# Autodesk Inventor assembly: Assembly2
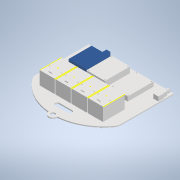
[picture p0: Inventor's stored thumbnail of the model, 180x180]
Saved by Autodesk Inventor 2020 (Build 240168000, 168)
## iProperties
Created: 2020-02-08
Part Number: Assembly2
Document SubType Name: Assembly
Designer: holtat
Author: holtat
## Documents named in this file (7)
- C:\Users\holtat\Documents\Inebriator\Assembly2.iam
- C:\Users\holtat\Documents\Inebriator\Top Plate.ipt
- C:\Users\holtat\Documents\Inebriator\Arduino.ipt
- C:\Users\holtat\Documents\Inebriator\ConnecterBoard.ipt
- C:\Users\holtat\Documents\Inebriator\Relay Board.ipt
- C:\Users\holtat\Documents\Inebriator\Plug.ipt
- C:\Users\holtat\Documents\Inebriator\Pump.ipt
## Components (9 placed, 6 different names)
1. Top Plate:1 — Mate:1, Mate:2, Mate:3, Mate:4, Mate:5, Mate:6, Flush:2, Flush:3, Flush:4, Flush:7, Mate:10, Flush:8, Mate:11, Flush:10
2. Arduino:1 — Mate:1, Flush:4, Mate:7, Flush:7
3. ConnecterBoard:1 — Mate:3, Flush:3, Mate:8
4. Relay Board:1 — Mate:2, Flush:2, Mate:7, Mate:8
5. Plug:1 — Mate:10, Flush:8
6. Pump:1 — Mate:6, Flush:6, Flush:9, Mate:13, Mate:14
7. Pump:2 — Mate:5, Flush:5, Flush:6, Mate:12, Flush:10
8. Pump:3 — Mate:4, Flush:5, Mate:12, Mate:13
9. Pump:4 — Mate:11, Flush:9, Mate:14
## Relationships (22: Mate 13, Flush 9)
- Mate:1: Top Plate:1 ↔ Arduino:1
- Mate:2: Top Plate:1 ↔ Relay Board:1
- Mate:3: Top Plate:1 ↔ ConnecterBoard:1
- Mate:4: Top Plate:1 ↔ Pump:3
- Mate:5: Top Plate:1 ↔ Pump:2
- Mate:6: Top Plate:1 ↔ Pump:1
- Flush:2 (12.7 mm): Top Plate:1 ↔ Relay Board:1
- Flush:3 (12.7 mm): Top Plate:1 ↔ ConnecterBoard:1
- Flush:4 (12.7 mm): Top Plate:1 ↔ Arduino:1
- Mate:7 (6.35 mm): Arduino:1 ↔ Relay Board:1
- Mate:8 (19.05 mm): ConnecterBoard:1 ↔ Relay Board:1
- Flush:5: Pump:2 ↔ Pump:3
- Flush:6: Pump:1 ↔ Pump:2
- Flush:7 (21.59 mm): Top Plate:1 ↔ Arduino:1
- Mate:10: Top Plate:1 ↔ Plug:1
- Flush:8 (2.54 mm): Top Plate:1 ↔ Plug:1
- Mate:11: Top Plate:1 ↔ Pump:4
- Flush:9: Pump:1 ↔ Pump:4
- Mate:12 (3.175 mm): Pump:2 ↔ Pump:3
- Mate:13 (3.175 mm): Pump:1 ↔ Pump:3
- Mate:14 (3.175 mm): Pump:1 ↔ Pump:4
- Flush:10 (32.8295 mm): Top Plate:1 ↔ Pump:2
